# Autodesk Inventor assembly: Back Funnel Frame
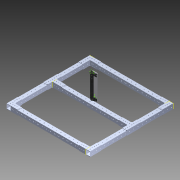
[picture p0: Inventor's stored thumbnail of the model, 180x180]
Saved by Autodesk Inventor 2014 (Build 180170000, 170)
## iProperties
Created: 2014-01-07
Part Number: Back Funnel Frame
Document SubType Name: Assembly
Designer: Michael
Mass: 644.134 g
Surface Area: 4249.21 cm^2
Volume: 237.688 cm^3
Density: 2.71 g/cm^3
Author: Michael
## Documents named in this file (7)
- C:\Users\Michael\Documents\Robotics\2014 Season\Funnel Catcher\Back Funnel Frame.iam
- C:\Users\Michael\Documents\Robotics\2014 Season\Funnel Catcher\Vex Pro 1x1 rectangular tubing 20 in length.ipt
- C:\Users\Michael\Documents\Robotics\2014 Season\Funnel Catcher\Vex Pro 1x1 rectangular tubing 18 in length.ipt
- C:\Users\Michael\Documents\Robotics\2014 Season\Funnel Catcher\Vex Pro 90 degree Gusset.ipt
- C:\Users\Michael\Documents\Robotics\2014 Season\Funnel Catcher\Vex Pro T Gusset.ipt
- C:\Users\Michael\Documents\Robotics\2014 Season\Funnel Catcher\9-16 in Pneumatic Cylinder (3 in Stroke).iam
- C:\Users\Michael\Documents\Robotics\2014 Season\Funnel Catcher\Flange for 3-4 in Piston.ipt
## Components (19 placed, 6 different names)
1. Vex Pro 1x1 rectangular tubing 20 in length:1 — Insert:1, Insert:2, Insert:13, Insert:15, Insert:16, Insert:17, Insert:19, Insert:20, Insert:32, Insert:33, Insert:40, Insert:41
2. Vex Pro 1x1 rectangular tubing 20 in length:2 — Insert:6, Insert:7, Insert:9, Insert:10, Insert:22, Insert:24, Insert:25, Insert:26, Insert:36, Insert:39, Insert:44, Insert:45
3. Vex Pro 1x1 rectangular tubing 18 in length:1 — Insert:11, Insert:12, Insert:14, Insert:21, Insert:23
4. Vex Pro 1x1 rectangular tubing 18 in length:2 — Insert:3, Insert:4, Insert:5, Insert:8, Insert:18, Insert:27
5. Vex Pro 90 degree Gusset:1 — Insert:1, Insert:2, Insert:3, Insert:4
6. Vex Pro 90 degree Gusset:2 — Insert:16, Insert:17, Insert:18
7. Vex Pro 90 degree Gusset:3 — Insert:5, Insert:6, Insert:7, Insert:8
8. Vex Pro 90 degree Gusset:4 — Insert:19, Insert:20, Insert:21
9. Vex Pro 90 degree Gusset:5 — Insert:25, Insert:26, Insert:27
10. Vex Pro 90 degree Gusset:6 — Insert:22, Insert:23, Insert:24
11. Vex Pro 90 degree Gusset:7 — Insert:13, Insert:14, Insert:15
12. Vex Pro 90 degree Gusset:8 — Insert:9, Insert:10, Insert:11, Insert:12
13. Vex Pro T Gusset:1 — Insert:32, Insert:33, Insert:34, Insert:35
14. Vex Pro T Gusset:2 — Insert:36, Insert:37, Insert:38, Insert:39
15. Vex Pro T Gusset:3 — Insert:40, Insert:41, Insert:42, Insert:43
16. Vex Pro T Gusset:4 — Insert:44, Insert:45, Insert:46, Insert:47
17. Vex Pro 1x1 rectangular tubing 18 in length:3 — Insert:34, Insert:35, Insert:37, Insert:38, Insert:42, Insert:43, Insert:46, Insert:47, Insert:50, Insert:51
18. Flange for 3-4 in Piston:1 — Insert:48, Insert:49, Insert:50, Insert:51
19. 9-16 in Pneumatic Cylinder (3 in Stroke):1 [sub-assembly] — Insert:48, Insert:49
## Relationships (47: Insert 47)
- Insert:1: Vex Pro 1x1 rectangular tubing 20 in length:1 ↔ Vex Pro 90 degree Gusset:1
- Insert:2: Vex Pro 1x1 rectangular tubing 20 in length:1 ↔ Vex Pro 90 degree Gusset:1
- Insert:3: Vex Pro 1x1 rectangular tubing 18 in length:2 ↔ Vex Pro 90 degree Gusset:1
- Insert:4: Vex Pro 1x1 rectangular tubing 18 in length:2 ↔ Vex Pro 90 degree Gusset:1
- Insert:5: Vex Pro 1x1 rectangular tubing 18 in length:2 ↔ Vex Pro 90 degree Gusset:3
- Insert:6: Vex Pro 1x1 rectangular tubing 20 in length:2 ↔ Vex Pro 90 degree Gusset:3
- Insert:7: Vex Pro 1x1 rectangular tubing 20 in length:2 ↔ Vex Pro 90 degree Gusset:3
- Insert:8: Vex Pro 1x1 rectangular tubing 18 in length:2 ↔ Vex Pro 90 degree Gusset:3
- Insert:9: Vex Pro 1x1 rectangular tubing 20 in length:2 ↔ Vex Pro 90 degree Gusset:8
- Insert:10: Vex Pro 1x1 rectangular tubing 20 in length:2 ↔ Vex Pro 90 degree Gusset:8
- Insert:11: Vex Pro 1x1 rectangular tubing 18 in length:1 ↔ Vex Pro 90 degree Gusset:8
- Insert:12: Vex Pro 1x1 rectangular tubing 18 in length:1 ↔ Vex Pro 90 degree Gusset:8
- Insert:13: Vex Pro 1x1 rectangular tubing 20 in length:1 ↔ Vex Pro 90 degree Gusset:7
- Insert:14: Vex Pro 1x1 rectangular tubing 18 in length:1 ↔ Vex Pro 90 degree Gusset:7
- Insert:15: Vex Pro 1x1 rectangular tubing 20 in length:1 ↔ Vex Pro 90 degree Gusset:7
- Insert:16: Vex Pro 1x1 rectangular tubing 20 in length:1 ↔ Vex Pro 90 degree Gusset:2
- Insert:17: Vex Pro 1x1 rectangular tubing 20 in length:1 ↔ Vex Pro 90 degree Gusset:2
- Insert:18: Vex Pro 1x1 rectangular tubing 18 in length:2 ↔ Vex Pro 90 degree Gusset:2
- Insert:19: Vex Pro 1x1 rectangular tubing 20 in length:1 ↔ Vex Pro 90 degree Gusset:4
- Insert:20: Vex Pro 1x1 rectangular tubing 20 in length:1 ↔ Vex Pro 90 degree Gusset:4
- Insert:21: Vex Pro 1x1 rectangular tubing 18 in length:1 ↔ Vex Pro 90 degree Gusset:4
- Insert:22: Vex Pro 1x1 rectangular tubing 20 in length:2 ↔ Vex Pro 90 degree Gusset:6
- Insert:23: Vex Pro 1x1 rectangular tubing 18 in length:1 ↔ Vex Pro 90 degree Gusset:6
- Insert:24: Vex Pro 1x1 rectangular tubing 20 in length:2 ↔ Vex Pro 90 degree Gusset:6
- Insert:25: Vex Pro 1x1 rectangular tubing 20 in length:2 ↔ Vex Pro 90 degree Gusset:5
- Insert:26: Vex Pro 1x1 rectangular tubing 20 in length:2 ↔ Vex Pro 90 degree Gusset:5
- Insert:27: Vex Pro 1x1 rectangular tubing 18 in length:2 ↔ Vex Pro 90 degree Gusset:5
- Insert:32: Vex Pro 1x1 rectangular tubing 20 in length:1 ↔ Vex Pro T Gusset:1
- Insert:33: Vex Pro 1x1 rectangular tubing 20 in length:1 ↔ Vex Pro T Gusset:1
- Insert:34: Vex Pro T Gusset:1 ↔ Vex Pro 1x1 rectangular tubing 18 in length:3
- Insert:35: Vex Pro T Gusset:1 ↔ Vex Pro 1x1 rectangular tubing 18 in length:3
- Insert:36: Vex Pro 1x1 rectangular tubing 20 in length:2 ↔ Vex Pro T Gusset:2
- Insert:37: Vex Pro T Gusset:2 ↔ Vex Pro 1x1 rectangular tubing 18 in length:3
- Insert:38: Vex Pro T Gusset:2 ↔ Vex Pro 1x1 rectangular tubing 18 in length:3
- Insert:39: Vex Pro 1x1 rectangular tubing 20 in length:2 ↔ Vex Pro T Gusset:2
- Insert:40: Vex Pro 1x1 rectangular tubing 20 in length:1 ↔ Vex Pro T Gusset:3
- Insert:41: Vex Pro 1x1 rectangular tubing 20 in length:1 ↔ Vex Pro T Gusset:3
- Insert:42: Vex Pro T Gusset:3 ↔ Vex Pro 1x1 rectangular tubing 18 in length:3
- Insert:43: Vex Pro T Gusset:3 ↔ Vex Pro 1x1 rectangular tubing 18 in length:3
- Insert:44: Vex Pro 1x1 rectangular tubing 20 in length:2 ↔ Vex Pro T Gusset:4
- Insert:45: Vex Pro 1x1 rectangular tubing 20 in length:2 ↔ Vex Pro T Gusset:4
- Insert:46: Vex Pro T Gusset:4 ↔ Vex Pro 1x1 rectangular tubing 18 in length:3
- Insert:47: Vex Pro T Gusset:4 ↔ Vex Pro 1x1 rectangular tubing 18 in length:3
- Insert:48: Flange for 3-4 in Piston:1 ↔ 9-16 in Pneumatic Cylinder (3 in Stroke):1
- Insert:49: Flange for 3-4 in Piston:1 ↔ 9-16 in Pneumatic Cylinder (3 in Stroke):1
- Insert:50: Vex Pro 1x1 rectangular tubing 18 in length:3 ↔ Flange for 3-4 in Piston:1
- Insert:51: Vex Pro 1x1 rectangular tubing 18 in length:3 ↔ Flange for 3-4 in Piston:1
